# Autodesk Inventor assembly: final_soft
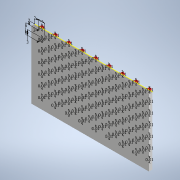
[picture p0: Inventor's stored thumbnail of the model, 180x180]
Saved by Autodesk Inventor 2020 (Build 240168000, 168)
## iProperties
Created: 2020-01-23
Part Number: final_soft
Document SubType Name: Assembly
Designer: sl65b
Author: sl65b
## Documents named in this file (4)
- C:\Users\sl65b\Desktop\Laboratory\MODEL\material_MK4\final_soft.iam
- C:\Users\sl65b\Desktop\Laboratory\MODEL\material_MK4\base_soft.ipt
- C:\Users\sl65b\Desktop\Laboratory\MODEL\material_MK4\soft_1.ipt
- C:\Users\sl65b\Desktop\Laboratory\MODEL\material_MK4\hard_1.ipt
## Components (223 placed, 3 different names)
1. base_soft:1 — Rigid:1, Rigid:2
2. soft_1:1 — Rigid:1, Rigid:3
3. soft_1:3
4. soft_1:4
5. soft_1:5
6. soft_1:6
7. soft_1:7
8. soft_1:8
9. soft_1:9
10. soft_1:10
11. soft_1:11
12. soft_1:12
13. soft_1:13
14. soft_1:14
15. soft_1:15
16. soft_1:16
17. soft_1:17
18. soft_1:18
19. soft_1:19
20. soft_1:20
21. soft_1:21
22. soft_1:22
23. soft_1:23
24. soft_1:24
25. soft_1:25
26. soft_1:26
27. soft_1:27
28. soft_1:28
29. soft_1:29
30. soft_1:30
31. soft_1:31
32. soft_1:32
33. soft_1:33
34. soft_1:34
35. soft_1:35
36. soft_1:36
37. soft_1:37
38. soft_1:38
39. soft_1:39
40. soft_1:40
41. soft_1:41
42. soft_1:42
43. soft_1:43
44. soft_1:44
45. soft_1:45
46. soft_1:46
47. soft_1:47
48. soft_1:48
49. soft_1:49
50. soft_1:50
51. soft_1:51
52. soft_1:52
53. soft_1:53
54. soft_1:54
55. soft_1:55
56. soft_1:56
57. soft_1:57
58. soft_1:58
59. soft_1:59
60. soft_1:60
61. soft_1:61
62. soft_1:62
63. soft_1:63
64. soft_1:64
65. soft_1:2 — Rigid:2, Rigid:4
66. soft_1:65
67. soft_1:66
68. soft_1:67
69. soft_1:68
70. soft_1:69
71. soft_1:70
72. soft_1:71
73. soft_1:72
74. soft_1:73
75. soft_1:74
76. soft_1:75
77. soft_1:76
78. soft_1:77
79. soft_1:78
80. soft_1:79
81. soft_1:80
82. soft_1:81
83. soft_1:82
84. soft_1:83
85. soft_1:84
86. soft_1:85
87. soft_1:86
88. soft_1:87
89. soft_1:88
90. soft_1:89
91. soft_1:90
92. soft_1:91
93. soft_1:92
94. soft_1:93
95. soft_1:94
96. soft_1:95
97. soft_1:96
98. soft_1:97
99. soft_1:98
100. soft_1:99
101. soft_1:100
102. soft_1:101
103. soft_1:102
104. soft_1:103
105. soft_1:104
106. soft_1:105
107. soft_1:106
108. soft_1:107
109. soft_1:108
110. soft_1:109
111. soft_1:110
112. soft_1:111
113. hard_1:1 — Rigid:3
114. hard_1:3
115. hard_1:4
116. hard_1:5
117. hard_1:6
118. hard_1:7
119. hard_1:8
120. hard_1:9
121. hard_1:10
122. hard_1:11
123. hard_1:12
124. hard_1:13
125. hard_1:14
126. hard_1:15
127. hard_1:16
128. hard_1:17
129. hard_1:18
130. hard_1:19
131. hard_1:20
132. hard_1:21
133. hard_1:22
134. hard_1:23
135. hard_1:24
136. hard_1:25
137. hard_1:26
138. hard_1:27
139. hard_1:28
140. hard_1:29
141. hard_1:30
142. hard_1:31
143. hard_1:32
144. hard_1:33
145. hard_1:34
146. hard_1:35
147. hard_1:36
148. hard_1:37
149. hard_1:38
150. hard_1:39
151. hard_1:40
152. hard_1:41
153. hard_1:42
154. hard_1:43
155. hard_1:44
156. hard_1:45
157. hard_1:46
158. hard_1:47
159. hard_1:48
160. hard_1:49
161. hard_1:50
162. hard_1:51
163. hard_1:52
164. hard_1:53
165. hard_1:54
166. hard_1:55
167. hard_1:56
168. hard_1:57
169. hard_1:58
170. hard_1:59
171. hard_1:60
172. hard_1:61
173. hard_1:62
174. hard_1:63
175. hard_1:64
176. hard_1:2 — Rigid:4
177. hard_1:65
178. hard_1:66
179. hard_1:67
180. hard_1:68
181. hard_1:69
182. hard_1:70
183. hard_1:71
184. hard_1:72
185. hard_1:73
186. hard_1:74
187. hard_1:75
188. hard_1:76
189. hard_1:77
190. hard_1:78
191. hard_1:79
192. hard_1:80
193. hard_1:81
194. hard_1:82
195. hard_1:83
196. hard_1:84
197. hard_1:85
198. hard_1:86
199. hard_1:87
200. hard_1:88
201. hard_1:89
202. hard_1:90
203. hard_1:91
204. hard_1:92
205. hard_1:93
206. hard_1:94
207. hard_1:95
208. hard_1:96
209. hard_1:97
210. hard_1:98
211. hard_1:99
212. hard_1:100
213. hard_1:101
214. hard_1:102
215. hard_1:103
216. hard_1:104
217. hard_1:105
218. hard_1:106
219. hard_1:107
220. hard_1:108
221. hard_1:109
222. hard_1:110
223. hard_1:111
## Component patterns: (63 elements, first: soft_1:1), (48 elements, first: soft_1:2), (63 elements, first: hard_1:1), (48 elements, first: hard_1:2)
## Relationships (4: WeldJoint 4)
- Rigid:1 [WeldJoint]: base_soft:1 ↔ soft_1:1
- Rigid:2 [WeldJoint]: base_soft:1 ↔ soft_1:2
- Rigid:3 [WeldJoint] (0.01 mm): soft_1:1 ↔ hard_1:1
- Rigid:4 [WeldJoint] (0.01 mm): soft_1:2 ↔ hard_1:2
